# Autodesk Inventor assembly: ShortElevatorFrame
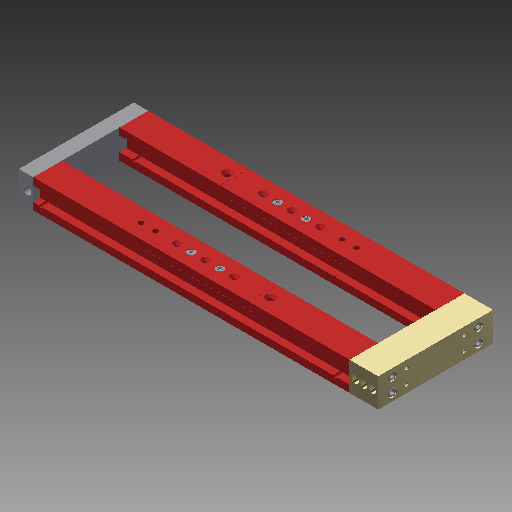
[picture p0: Inventor's stored thumbnail of the model, 512x512]
Saved by Autodesk Inventor 2019 (Build 230136000, 136)
## iProperties
Created: 2019-09-28
Part Number: ShortElevatorFrame
Document SubType Name: Assembly
Designer: james
Author: james
## Documents named in this file (4)
- F:\JimsDesign\Jims2020FTC\ShortElevatorFrame.iam
- F:\JimsDesign\Jims2020FTC\ElvatorEnd.iam
- F:\JimsDesign\Jims2020FTC\ElvatorBottom.iam
- F:\JimsDesign\Jims2020FTC\EvelShortBackBeam.iam
## Components (4 placed, 3 different names)
1. ElvatorBottom:1 [sub-assembly] — Mate:1, Mate:2, Mate:3, Mate:4, Mate:5, Mate:6
2. ElvatorEnd:2 [sub-assembly] — Mate:7, Mate:8, Mate:9
3. EvelShortBackBeam:1 [sub-assembly] — Mate:1, Mate:2, Mate:3, Mate:7
4. EvelShortBackBeam:2 [sub-assembly] — Mate:4, Mate:5, Mate:6, Mate:8, Mate:9
## Relationships (9: Mate 9)
- Mate:1: ElvatorBottom:1 ↔ EvelShortBackBeam:1
- Mate:2: ElvatorBottom:1 ↔ EvelShortBackBeam:1
- Mate:3: ElvatorBottom:1 ↔ EvelShortBackBeam:1
- Mate:4: ElvatorBottom:1 ↔ EvelShortBackBeam:2
- Mate:5: ElvatorBottom:1 ↔ EvelShortBackBeam:2
- Mate:6: ElvatorBottom:1 ↔ EvelShortBackBeam:2
- Mate:7: ElvatorEnd:2 ↔ EvelShortBackBeam:1
- Mate:8: ElvatorEnd:2 ↔ EvelShortBackBeam:2
- Mate:9: ElvatorEnd:2 ↔ EvelShortBackBeam:2
